# Autodesk Inventor assembly: ElvFixedFrame
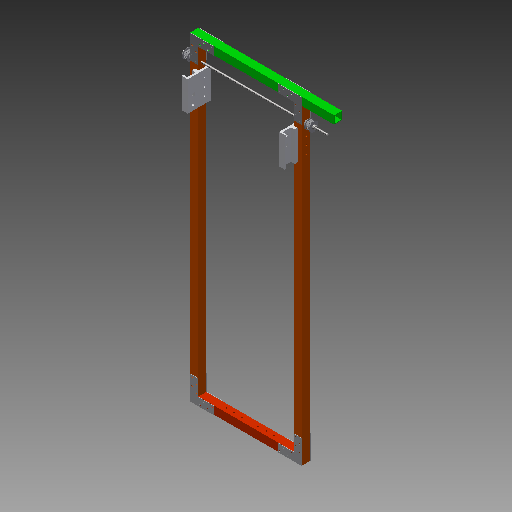
[picture p0: Inventor's stored thumbnail of the model, 512x512]
Saved by Autodesk Inventor 2019 (Build 230136000, 136)
## iProperties
Created: 2019-01-10
Part Number: ElvFixedFrame
Document SubType Name: Assembly
Designer: james
Mass: 1496.37 g
Surface Area: 5918.16 cm^2
Volume: 572.084 cm^3
Density: 2.61565 g/cm^3
Author: james
## Documents named in this file (7)
- F:\JimsDesign\2019CHS4089\ElvFixedFrame.iam
- F:\JimsDesign\2019CHS4089\ElvCrossBeam.ipt
- F:\JimsDesign\2019CHS4089\ElvFixedBeam.ipt
- F:\JimsDesign\2019CHS4089\ElvShaft.iam
- F:\JimsDesign\2019CHS4089\ElvTopBeam.ipt
- F:\JimsDesign\2019CHS4089\elvRivetPlate.ipt
- F:\JimsDesign\2019CHS4089\ElvDelV5.ipt
## Components (15 placed, 6 different names)
1. ElvCrossBeam:1 — Mate:34, Mate:35, Mate:36, Mate:38, Mate:43, Mate:44, Mate:47, Mate:48, Mate:49
2. ElvFixedBeam:1 — Flush:6, Flush:7, Mate:14, Mate:19, Flush:9, Mate:25, Flush:12, Mate:26, Mate:27, Mate:37, Mate:39, Mate:40, Mate:41, Mate:42, Mate:46
3. ElvFixedBeam:2 — Mate:13, Flush:5, Mate:21, Mate:22, Mate:28, Mate:29, Mate:30, Mate:31, Mate:32, Mate:33, Mate:45, Mate:50, Mate:51, Mate:52
4. ElvDelV5:1 — Mate:26, Mate:27, Mate:46
5. ElvDelV5:2 — Mate:21, Mate:22, Mate:45
6. ElvShaft:1 [sub-assembly] — Mate:19
7. ElvTopBeam:1 — Mate:13, Flush:5, Flush:6, Flush:7, Mate:14, Mate:23, Flush:8
8. elvRivetPlate:1 — Mate:23, Flush:8, Flush:9
9. elvRivetPlate:2 — Mate:39, Mate:40, Mate:41
10. elvRivetPlate:3 — Mate:25, Flush:12, Mate:37, Mate:38
11. elvRivetPlate:4 — Mate:28, Mate:29, Mate:30
12. elvRivetPlate:5 — Mate:31, Mate:32, Mate:33, Mate:34, Mate:35, Mate:36
13. elvRivetPlate:6 — Mate:42, Mate:43, Mate:44
14. elvRivetPlate:7 — Mate:50, Mate:51, Mate:52
15. elvRivetPlate:8 — Mate:47, Mate:48, Mate:49
## Relationships (40: Mate 34, Flush 6)
- Mate:13: ElvFixedBeam:2 ↔ ElvTopBeam:1
- Flush:5: ElvFixedBeam:2 ↔ ElvTopBeam:1
- Flush:6: ElvFixedBeam:1 ↔ ElvTopBeam:1
- Flush:7: ElvFixedBeam:1 ↔ ElvTopBeam:1
- Mate:14: ElvFixedBeam:1 ↔ ElvTopBeam:1
- Mate:19: ElvFixedBeam:1 ↔ ElvShaft:1
- Mate:21: ElvFixedBeam:2 ↔ ElvDelV5:2
- Mate:22: ElvFixedBeam:2 ↔ ElvDelV5:2
- Mate:23: ElvTopBeam:1 ↔ elvRivetPlate:1
- Flush:8: ElvTopBeam:1 ↔ elvRivetPlate:1
- Flush:9: ElvFixedBeam:1 ↔ elvRivetPlate:1
- Mate:25: ElvFixedBeam:1 ↔ elvRivetPlate:3
- Flush:12: ElvFixedBeam:1 ↔ elvRivetPlate:3
- Mate:26: ElvFixedBeam:1 ↔ ElvDelV5:1
- Mate:27: ElvFixedBeam:1 ↔ ElvDelV5:1
- Mate:28: ElvFixedBeam:2 ↔ elvRivetPlate:4
- Mate:29: ElvFixedBeam:2 ↔ elvRivetPlate:4
- Mate:30: ElvFixedBeam:2 ↔ elvRivetPlate:4
- Mate:31: ElvFixedBeam:2 ↔ elvRivetPlate:5
- Mate:32: ElvFixedBeam:2 ↔ elvRivetPlate:5
- Mate:33: ElvFixedBeam:2 ↔ elvRivetPlate:5
- Mate:34: ElvCrossBeam:1 ↔ elvRivetPlate:5
- Mate:35: ElvCrossBeam:1 ↔ elvRivetPlate:5
- Mate:36: ElvCrossBeam:1 ↔ elvRivetPlate:5
- Mate:37: ElvFixedBeam:1 ↔ elvRivetPlate:3
- Mate:38: ElvCrossBeam:1 ↔ elvRivetPlate:3
- Mate:39: ElvFixedBeam:1 ↔ elvRivetPlate:2
- Mate:40: ElvFixedBeam:1 ↔ elvRivetPlate:2
- Mate:41: ElvFixedBeam:1 ↔ elvRivetPlate:2
- Mate:42: ElvFixedBeam:1 ↔ elvRivetPlate:6
- Mate:43: ElvCrossBeam:1 ↔ elvRivetPlate:6
- Mate:44: ElvCrossBeam:1 ↔ elvRivetPlate:6
- Mate:45: ElvFixedBeam:2 ↔ ElvDelV5:2
- Mate:46: ElvFixedBeam:1 ↔ ElvDelV5:1
- Mate:47: ElvCrossBeam:1 ↔ elvRivetPlate:8
- Mate:48: ElvCrossBeam:1 ↔ elvRivetPlate:8
- Mate:49: ElvCrossBeam:1 ↔ elvRivetPlate:8
- Mate:50: ElvFixedBeam:2 ↔ elvRivetPlate:7
- Mate:51: ElvFixedBeam:2 ↔ elvRivetPlate:7
- Mate:52: ElvFixedBeam:2 ↔ elvRivetPlate:7
